# Autodesk Inventor assembly: MainStanokLathe
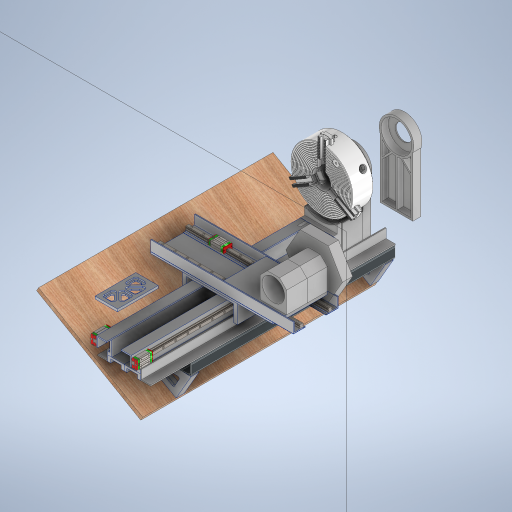
[picture p0: Inventor's stored thumbnail of the model, 512x512]
Saved by Autodesk Inventor 2024 (Build 280153000, 153)
## iProperties
Created: 2023-08-15
Part Number: MainStanokLathe
Document SubType Name: Assembly
Designer: Kippi
Mass: 47808.8 g
Surface Area: 40542.6 cm^2
Volume: 14656.1 cm^3
Density: 3.26205 g/cm^3
Author: Kippi
## Documents named in this file (13)
- C:\WorkProject\CNC_Lathe\MainStanokLathe.iam
- C:\WorkProject\CNC_Lathe\Stanina.iam
- C:\WorkProject\CNC_Lathe\YaxisAss.iam
- C:\WorkProject\CNC_Lathe\Rails\HGR20R LINEAR GUIDE RAIL, CONFIGURABLE, 1000 mm.ipt
- C:\WorkProject\CNC_Lathe\Rails\HGH20CAZ0C, BLOCK, MIDSECTION.ipt
- C:\WorkProject\CNC_Lathe\Podkladka.ipt
- C:\WorkProject\CNC_Lathe\FlanecForwardBabka.ipt
- C:\WorkProject\CNC_Lathe\Babka.iam
- C:\WorkProject\CNC_Lathe\KaretkaYaxis.ipt
- C:\WorkProject\CNC_Lathe\ProkladkaA.ipt
- C:\WorkProject\CNC_Lathe\KorpusOsnova.ipt
- C:\WorkProject\CNC_Lathe\OsnovaBaraban.ipt
- C:\WorkProject\CNC_Lathe\InstruumentarBaraban.ipt
## Components (16 placed, 12 different names)
1. Stanina:1 [sub-assembly] — Flush:7, Mate:21, Mate:24, Mate:25, Mate:26, Mate:34, Mate:35, Flush:10, Flush:11, Mate:38, Mate:39, Mate:43
2. YaxisAss:1 [sub-assembly] — Mate:13, Mate:14, Mate:19, Mate:42, Flush:12
3. HGH20CAZ0C, BLOCK, MIDSECTION:5 — Mate:13, Mate:14, Mate:20
4. FlanecForwardBabka:1 — Flush:7, Mate:22, Flush:8
5. KaretkaYaxis:2 — Mate:19, Mate:20, Mate:27, Flush:9, Mate:28, Mate:30
6. Babka:2 [sub-assembly] — Mate:23, Mate:24
7. ProkladkaA:2 — Mate:21, Mate:22, Flush:8, Mate:23
8. KorpusOsnova:2 — Mate:25, Mate:26
9. OsnovaBaraban:1 — Mate:27, Flush:9, Mate:28, Mate:29, Mate:31, Mate:32
10. OsnovaBaraban:2 — Mate:29, Mate:30, Mate:31, Mate:33
11. InstruumentarBaraban:2 — Mate:32, Mate:33
12. HGR20R LINEAR GUIDE RAIL, CONFIGURABLE, 1000 mm:3 — Mate:35, Flush:10, Mate:36, Mate:37, Mate:38
13. HGR20R LINEAR GUIDE RAIL, CONFIGURABLE, 1000 mm:4 — Mate:34, Flush:11, Mate:39, Mate:40, Mate:41
14. HGH20CAZ0C, BLOCK, MIDSECTION:8 — Mate:40, Mate:41, Mate:44
15. HGH20CAZ0C, BLOCK, MIDSECTION:9 — Mate:36, Mate:37
16. Podkladka:2 — Mate:42, Flush:12, Mate:43, Mate:44
## Relationships (34: Mate 28, Flush 6)
- Mate:13: YaxisAss:1 ↔ HGH20CAZ0C, BLOCK, MIDSECTION:5
- Mate:14: YaxisAss:1 ↔ HGH20CAZ0C, BLOCK, MIDSECTION:5
- Flush:7: Stanina:1 ↔ FlanecForwardBabka:1
- Mate:19: YaxisAss:1 ↔ KaretkaYaxis:2
- Mate:20: HGH20CAZ0C, BLOCK, MIDSECTION:5 ↔ KaretkaYaxis:2
- Mate:21: Stanina:1 ↔ ProkladkaA:2
- Mate:22: FlanecForwardBabka:1 ↔ ProkladkaA:2
- Flush:8: FlanecForwardBabka:1 ↔ ProkladkaA:2
- Mate:23: Babka:2 ↔ ProkladkaA:2
- Mate:24: Stanina:1 ↔ Babka:2
- Mate:25: Stanina:1 ↔ KorpusOsnova:2
- Mate:26: Stanina:1 ↔ KorpusOsnova:2
- Mate:27: KaretkaYaxis:2 ↔ OsnovaBaraban:1
- Flush:9: KaretkaYaxis:2 ↔ OsnovaBaraban:1
- Mate:28: KaretkaYaxis:2 ↔ OsnovaBaraban:1
- Mate:29: OsnovaBaraban:1 ↔ OsnovaBaraban:2
- Mate:30: KaretkaYaxis:2 ↔ OsnovaBaraban:2
- Mate:31: OsnovaBaraban:1 ↔ OsnovaBaraban:2
- Mate:32: OsnovaBaraban:1 ↔ InstruumentarBaraban:2
- Mate:33: OsnovaBaraban:2 ↔ InstruumentarBaraban:2
- Mate:34: Stanina:1 ↔ HGR20R LINEAR GUIDE RAIL, CONFIGURABLE, 1000 mm:4
- Mate:35: Stanina:1 ↔ HGR20R LINEAR GUIDE RAIL, CONFIGURABLE, 1000 mm:3
- Flush:10: Stanina:1 ↔ HGR20R LINEAR GUIDE RAIL, CONFIGURABLE, 1000 mm:3
- Flush:11: Stanina:1 ↔ HGR20R LINEAR GUIDE RAIL, CONFIGURABLE, 1000 mm:4
- Mate:36: HGR20R LINEAR GUIDE RAIL, CONFIGURABLE, 1000 mm:3 ↔ HGH20CAZ0C, BLOCK, MIDSECTION:9
- Mate:37: HGR20R LINEAR GUIDE RAIL, CONFIGURABLE, 1000 mm:3 ↔ HGH20CAZ0C, BLOCK, MIDSECTION:9
- Mate:38: Stanina:1 ↔ HGR20R LINEAR GUIDE RAIL, CONFIGURABLE, 1000 mm:3
- Mate:39: Stanina:1 ↔ HGR20R LINEAR GUIDE RAIL, CONFIGURABLE, 1000 mm:4
- Mate:40: HGR20R LINEAR GUIDE RAIL, CONFIGURABLE, 1000 mm:4 ↔ HGH20CAZ0C, BLOCK, MIDSECTION:8
- Mate:41: HGR20R LINEAR GUIDE RAIL, CONFIGURABLE, 1000 mm:4 ↔ HGH20CAZ0C, BLOCK, MIDSECTION:8
- Mate:42: YaxisAss:1 ↔ Podkladka:2
- Flush:12: YaxisAss:1 ↔ Podkladka:2
- Mate:43: Stanina:1 ↔ Podkladka:2
- Mate:44: HGH20CAZ0C, BLOCK, MIDSECTION:8 ↔ Podkladka:2
